# Autodesk Inventor assembly: Flipper Chain Drive
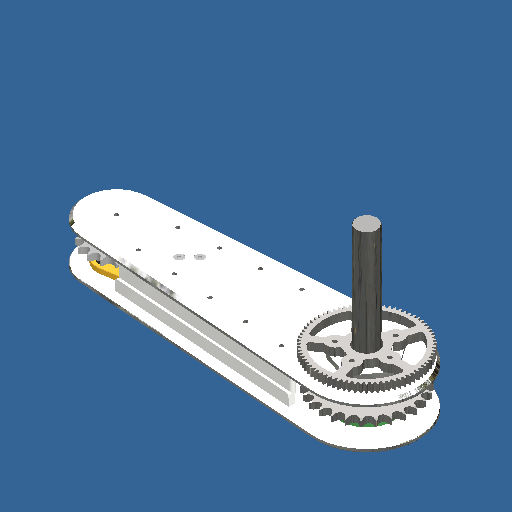
[picture p0: Inventor's stored thumbnail of the model, 512x512]
Saved by Autodesk Inventor 2023 (Build 270158030, 158C)
## iProperties
Created: 2023-01-21
Part Number: Flipper Chain Drive
Document SubType Name: Assembly
Designer: AdminForWorker
Title: Flipper Chain Drive v35
Author: AdminForWorker
## Documents named in this file (30)
- C:\Users\kumpu\Documents\SBU\CAD\SBRT\Robocup Rescue\Drive\v1\Flipper\Flipper Chain Drive.iam
- C:\Users\kumpu\Documents\SBU\CAD\SBRT\Robocup Rescue\Drive\v1\Flipper\Idler Sprocket 16t v12.iam
- C:\Users\kumpu\Documents\SBU\CAD\SBRT\Robocup Rescue\Drive\v1\Flipper\27t track drive sprocket v25.iam
- C:\Users\kumpu\Documents\SBU\CAD\SBRT\Robocup Rescue\Drive\v1\Flipper\chain_male v7.ipt
- C:\Users\kumpu\Documents\SBU\CAD\SBRT\Robocup Rescue\Drive\v1\Flipper\chain_female v7.ipt
- C:\Users\kumpu\Documents\SBU\CAD\SBRT\Robocup Rescue\Drive\v1\Flipper\98585A121_Heavy Duty External Retaining Ring v2.ipt
- C:\Users\kumpu\Documents\SBU\CAD\SBRT\Robocup Rescue\Drive\v1\Flipper\94328A911_Black Oxide Alloy Steel Low-Profile Shoulder Screw v2.ipt
- C:\Users\kumpu\Documents\SBU\CAD\SBRT\Robocup Rescue\Drive\v1\Flipper\2868T199_High-Load Oil-Embedded 863 Sleeve Bearing (1) v2.ipt
- C:\Users\kumpu\Documents\SBU\CAD\SBRT\Robocup Rescue\Drive\v1\Flipper\91263A553_Zinc-Plated Alloy Steel Hex Drive Flat Head Screw v1.ipt
- C:\Users\kumpu\Documents\SBU\CAD\SBRT\Robocup Rescue\Drive\v1\Flipper\outisde panel.ipt
- C:\Users\kumpu\Documents\SBU\CAD\SBRT\Robocup Rescue\Drive\v1\Flipper\outside panel bushing support.ipt
- C:\Users\kumpu\Documents\SBU\CAD\SBRT\Robocup Rescue\Drive\v1\Flipper\98585A121_Heavy Duty External Retaining Ring v2(Mirror).ipt
- C:\Users\kumpu\Documents\SBU\CAD\SBRT\Robocup Rescue\Drive\v1\Flipper\2868T199_High-Load Oil-Embedded 863 Sleeve Bearing (1) v2(Mirror).ipt
- C:\Users\kumpu\Documents\SBU\CAD\SBRT\Robocup Rescue\Drive\v1\Flipper\inside panel.ipt
- C:\Users\kumpu\Documents\SBU\CAD\SBRT\Robocup Rescue\Drive\v1\Flipper\inside panel bushing support.ipt
- C:\Users\kumpu\Documents\SBU\CAD\SBRT\Robocup Rescue\Drive\v1\Flipper\91253A245_Black-Oxide Alloy Steel Hex Drive Flat Head Screw v1.ipt
- C:\Users\kumpu\Documents\SBU\CAD\SBRT\Robocup Rescue\Drive\v1\Flipper\90128A229_Zinc-Plated Alloy Steel Socket Head Screw (1) v1.ipt
- C:\Users\kumpu\Documents\SBU\CAD\SBRT\Robocup Rescue\Drive\v1\Flipper\M4x8 BHCS v1(Mirror).ipt
- C:\Users\kumpu\Documents\SBU\CAD\SBRT\Robocup Rescue\Drive\v1\Flipper\top chain glide.ipt
- C:\Users\kumpu\Documents\SBU\CAD\SBRT\Robocup Rescue\Drive\v1\Flipper\bottom chain glide.ipt
- C:\Users\kumpu\Documents\SBU\CAD\SBRT\Robocup Rescue\Drive\v1\Flipper\tensioner washer.ipt
- C:\Users\kumpu\Documents\SBU\CAD\SBRT\Robocup Rescue\Drive\v1\Flipper\tensioner anchor block.ipt
- C:\Users\kumpu\Documents\SBU\CAD\SBRT\Robocup Rescue\Drive\v1\Flipper\tensioner inside plate.ipt
- C:\Users\kumpu\Documents\SBU\CAD\SBRT\Robocup Rescue\Drive\v1\Flipper\tensioner spacer.ipt
- C:\Users\kumpu\Documents\SBU\CAD\SBRT\Robocup Rescue\Drive\v1\Flipper\tensioner mobile block.ipt
- C:\Users\kumpu\Documents\SBU\CAD\SBRT\Robocup Rescue\Drive\v1\Flipper\tensioner outside plate.ipt
- C:\Users\kumpu\Documents\SBU\CAD\SBRT\Robocup Rescue\Drive\v1\Flipper\Idler Shaft.ipt
- C:\Users\kumpu\Documents\SBU\CAD\SBRT\Robocup Rescue\Drive\v1\Flipper\Drive Shaft.ipt
- C:\Users\kumpu\Documents\SBU\CAD\SBRT\Robocup Rescue\Drive\v1\Flipper\Spur Gear (74 teeth).ipt
- C:\Users\kumpu\Documents\SBU\CAD\SBRT\Robocup Rescue\Drive\v1\Flipper\gearSpacer.ipt
## Components (111 placed, 29 different names)
1. Idler Sprocket 16t v12:1 [sub-assembly]
2. 27t track drive sprocket v25:1 [sub-assembly]
3. 98585A121_Heavy Duty External Retaining Ring v2:1
4. 94328A911_Black Oxide Alloy Steel Low-Profile Shoulder Screw v2:1
5. 2868T199_High-Load Oil-Embedded 863 Sleeve Bearing (1) v2:1
6. 91263A553_Zinc-Plated Alloy Steel Hex Drive Flat Head Screw v1:1
7. 91263A553_Zinc-Plated Alloy Steel Hex Drive Flat Head Screw v1:2
8. 91263A553_Zinc-Plated Alloy Steel Hex Drive Flat Head Screw v1:3
9. 91263A553_Zinc-Plated Alloy Steel Hex Drive Flat Head Screw v1:4
10. 91263A553_Zinc-Plated Alloy Steel Hex Drive Flat Head Screw v1:5
11. outisde panel:1 — Insert:5, Insert:6
12. outside panel bushing support:1
13. 98585A121_Heavy Duty External Retaining Ring v2:2
14. 98585A121_Heavy Duty External Retaining Ring v2(Mirror):1
15. 98585A121_Heavy Duty External Retaining Ring v2(Mirror):2
16. 2868T199_High-Load Oil-Embedded 863 Sleeve Bearing (1) v2(Mirror):1
17. inside panel:1 — Mate:2, Mate:3, Insert:1, Insert:2, Insert:3, Insert:4, Insert:7
18. inside panel bushing support:1
19. 91253A245_Black-Oxide Alloy Steel Hex Drive Flat Head Screw v1:1
20. 91253A245_Black-Oxide Alloy Steel Hex Drive Flat Head Screw v1:2
21. 91253A245_Black-Oxide Alloy Steel Hex Drive Flat Head Screw v1:3
22. 91253A245_Black-Oxide Alloy Steel Hex Drive Flat Head Screw v1:4
23. 90128A229_Zinc-Plated Alloy Steel Socket Head Screw (1) v1:1
24. 90128A229_Zinc-Plated Alloy Steel Socket Head Screw (1) v1:2
25. 91253A245_Black-Oxide Alloy Steel Hex Drive Flat Head Screw v1:5
26. 91253A245_Black-Oxide Alloy Steel Hex Drive Flat Head Screw v1:6
27. 91253A245_Black-Oxide Alloy Steel Hex Drive Flat Head Screw v1:7
28. 91253A245_Black-Oxide Alloy Steel Hex Drive Flat Head Screw v1:8
29. M4x8 BHCS v1(Mirror):1
30. M4x8 BHCS v1(Mirror):2
31. top chain glide:1 — Insert:3, Insert:4, Insert:6
32. bottom chain glide:1 — Insert:1, Insert:2, Insert:5
33. tensioner washer:1
34. tensioner anchor block:1
35. tensioner inside plate:1
36. tensioner spacer:1
37. tensioner mobile block:1
38. tensioner outside plate:1
39. Idler Shaft:1
40. Drive Shaft:1 — Mate:1, Mate:3
41. Spur Gear (74 teeth):1 — Mate:1, Mate:2, Insert:7, Insert:8, Mate:4
42. gearSpacer:1 — Insert:8, Mate:4
43. chain_female v7:7
44. chain_female v7:6
45. chain_female v7:5
46. chain_female v7:4
47. chain_female v7:3
48. chain_female v7:2
49. chain_female v7:1
50. chain_female v7:8
51. chain_female v7:20
52. chain_female v7:32
53. chain_female v7:33
54. chain_female v7:34
55. chain_female v7:111
56. chain_female v7:110
57. chain_female v7:109
58. chain_female v7:108
59. chain_female v7:107
60. chain_female v7:106
61. chain_female v7:105
62. chain_female v7:104
63. chain_female v7:103
64. chain_female v7:102
65. chain_female v7:101
66. chain_female v7:115
67. chain_female v7:114
68. chain_female v7:113
69. chain_female v7:112
70. chain_female v7:116
71. chain_female v7:117
72. chain_female v7:118
73. chain_female v7:119
74. chain_female v7:120
75. chain_female v7:122
76. chain_female v7:121
77. chain_male v7:1
78. chain_male v7:2
79. chain_male v7:3
80. chain_male v7:4
81. chain_male v7:5
82. chain_male v7:6
83. chain_male v7:7
84. chain_male v7:19
85. chain_male v7:20
86. chain_male v7:32
87. chain_male v7:33
88. chain_male v7:34
89. chain_male v7:35
90. chain_male v7:102
91. chain_male v7:103
92. chain_male v7:104
93. chain_male v7:105
94. chain_male v7:106
95. chain_male v7:107
96. chain_male v7:108
97. chain_male v7:109
98. chain_male v7:110
99. chain_male v7:111
100. chain_male v7:112
101. chain_male v7:113
102. chain_male v7:114
103. chain_male v7:115
104. chain_male v7:116
105. chain_male v7:117
106. chain_male v7:118
107. chain_male v7:119
108. chain_male v7:120
109. chain_male v7:121
110. chain_male v7:122
111. chain_male v7:123
## Relationships (12: Insert 8, Mate 4)
- Mate:1: Drive Shaft:1 ↔ Spur Gear (74 teeth):1
- Mate:2: inside panel:1 ↔ Spur Gear (74 teeth):1
- Mate:3: inside panel:1 ↔ Drive Shaft:1
- Insert:1: inside panel:1 ↔ bottom chain glide:1
- Insert:2: inside panel:1 ↔ bottom chain glide:1
- Insert:3: inside panel:1 ↔ top chain glide:1
- Insert:4: inside panel:1 ↔ top chain glide:1
- Insert:5: outisde panel:1 ↔ bottom chain glide:1
- Insert:6: outisde panel:1 ↔ top chain glide:1
- Insert:7 (6.35 mm): inside panel:1 ↔ Spur Gear (74 teeth):1
- Insert:8: Spur Gear (74 teeth):1 ↔ gearSpacer:1
- Mate:4: Spur Gear (74 teeth):1 ↔ gearSpacer:1
